# Autodesk Inventor assembly: Hopper Motor Holder assy
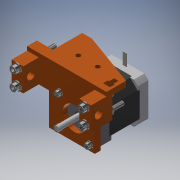
[picture p0: Inventor's stored thumbnail of the model, 180x180]
Saved by Autodesk Inventor 2018 (Build 220112000, 112)
## iProperties
Created: 2017-09-26
Part Number: Hopper Motor Holder assy
Document SubType Name: Assembly
Designer: Gabriel Smolnycki
Author: Gabriel Smolnycki
## Documents named in this file (9)
- H:\dev\planb\mechanics\V1INV\Subassemblies\Hopper Motor Holder assy.iam
- H:\dev\planb\mechanics\V1INV\Hopper\Hopper Motor Holder.ipt
- H:\dev\planb\mechanics\V1INV\Hopper\Hopper Smooth Rod Clamp.ipt
- H:\dev\planb\mechanics\V1INV\Hardware\M4x40 SS SHCS.ipt
- H:\dev\planb\mechanics\V1INV\Hardware\M4 SS Washer.ipt
- H:\dev\planb\mechanics\V1INV\Hardware\M4 SS Locknut.ipt
- H:\dev\planb\mechanics\V1INV\Electronics\ST4118L1804-B.ipt
- H:\dev\planb\mechanics\V1INV\Hardware\M3 SS Washer.ipt
- H:\dev\planb\mechanics\V1INV\Hardware\M3x10 SS SHCS.ipt
## Components (28 placed, 8 different names)
1. Hopper Motor Holder:1 — Insert:1, Insert:2, Insert:5, Insert:6, Insert:17, Insert:18, Mate:1, Insert:19, Insert:20, Insert:23, Insert:24, Insert:25, Insert:26, Insert:27, Insert:28
2. Hopper Smooth Rod Clamp:1 — Insert:1, Insert:2, Insert:3, Insert:4
3. Hopper Smooth Rod Clamp:2 — Insert:3, Insert:4, Insert:13, Insert:14
4. Hopper Smooth Rod Clamp:3 — Insert:5, Insert:6, Insert:7, Insert:8
5. Hopper Smooth Rod Clamp:4 — Insert:7, Insert:8, Insert:9, Insert:10
6. M4x40 SS SHCS:1 — Insert:16
7. M4x40 SS SHCS:2 — Insert:15
8. M4x40 SS SHCS:3 — Insert:12
9. M4x40 SS SHCS:4 — Insert:11
10. M4 SS Washer:1 — Insert:9, Insert:11
11. M4 SS Washer:2 — Insert:10, Insert:12
12. M4 SS Washer:3 — Insert:13, Insert:15
13. M4 SS Washer:4 — Insert:14, Insert:16
14. M4 SS Locknut:1 — Insert:17, Mate:1
15. M4 SS Locknut:2 — Insert:18
16. M4 SS Washer:5 — Insert:19, Insert:21
17. M4 SS Washer:6 — Insert:20, Insert:22
18. M4 SS Locknut:3 — Insert:21
19. M4 SS Locknut:4 — Insert:22
20. ST4118L1804-B:1 — Insert:23, Insert:24
21. M3 SS Washer:1 — Insert:25, Insert:29
22. M3 SS Washer:2 — Insert:26, Insert:31
23. M3 SS Washer:3 — Insert:27, Insert:30
24. M3 SS Washer:4 — Insert:28, Insert:32
25. M3x10 SS SHCS:1 — Insert:29
26. M3x10 SS SHCS:2 — Insert:30
27. M3x10 SS SHCS:3 — Insert:31
28. M3x10 SS SHCS:4 — Insert:32
## Relationships (33: Insert 32, Mate 1)
- Insert:1: Hopper Motor Holder:1 ↔ Hopper Smooth Rod Clamp:1
- Insert:2: Hopper Motor Holder:1 ↔ Hopper Smooth Rod Clamp:1
- Insert:3: Hopper Smooth Rod Clamp:1 ↔ Hopper Smooth Rod Clamp:2
- Insert:4: Hopper Smooth Rod Clamp:1 ↔ Hopper Smooth Rod Clamp:2
- Insert:5: Hopper Motor Holder:1 ↔ Hopper Smooth Rod Clamp:3
- Insert:6: Hopper Motor Holder:1 ↔ Hopper Smooth Rod Clamp:3
- Insert:7: Hopper Smooth Rod Clamp:3 ↔ Hopper Smooth Rod Clamp:4
- Insert:8: Hopper Smooth Rod Clamp:3 ↔ Hopper Smooth Rod Clamp:4
- Insert:9: Hopper Smooth Rod Clamp:4 ↔ M4 SS Washer:1
- Insert:10: Hopper Smooth Rod Clamp:4 ↔ M4 SS Washer:2
- Insert:11: M4x40 SS SHCS:4 ↔ M4 SS Washer:1
- Insert:12: M4x40 SS SHCS:3 ↔ M4 SS Washer:2
- Insert:13: Hopper Smooth Rod Clamp:2 ↔ M4 SS Washer:3
- Insert:14: Hopper Smooth Rod Clamp:2 ↔ M4 SS Washer:4
- Insert:15: M4x40 SS SHCS:2 ↔ M4 SS Washer:3
- Insert:16: M4x40 SS SHCS:1 ↔ M4 SS Washer:4
- Insert:17: Hopper Motor Holder:1 ↔ M4 SS Locknut:1
- Insert:18: Hopper Motor Holder:1 ↔ M4 SS Locknut:2
- Mate:1: Hopper Motor Holder:1 ↔ M4 SS Locknut:1
- Insert:19: Hopper Motor Holder:1 ↔ M4 SS Washer:5
- Insert:20: Hopper Motor Holder:1 ↔ M4 SS Washer:6
- Insert:21: M4 SS Washer:5 ↔ M4 SS Locknut:3
- Insert:22: M4 SS Washer:6 ↔ M4 SS Locknut:4
- Insert:23: Hopper Motor Holder:1 ↔ ST4118L1804-B:1
- Insert:24: Hopper Motor Holder:1 ↔ ST4118L1804-B:1
- Insert:25: Hopper Motor Holder:1 ↔ M3 SS Washer:1
- Insert:26: Hopper Motor Holder:1 ↔ M3 SS Washer:2
- Insert:27: Hopper Motor Holder:1 ↔ M3 SS Washer:3
- Insert:28: Hopper Motor Holder:1 ↔ M3 SS Washer:4
- Insert:29: M3 SS Washer:1 ↔ M3x10 SS SHCS:1
- Insert:30: M3 SS Washer:3 ↔ M3x10 SS SHCS:2
- Insert:31: M3 SS Washer:2 ↔ M3x10 SS SHCS:3
- Insert:32: M3 SS Washer:4 ↔ M3x10 SS SHCS:4
